# Autodesk Inventor assembly: full
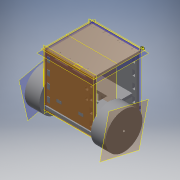
[picture p0: Inventor's stored thumbnail of the model, 180x180]
Saved by Autodesk Inventor 2018 (Build 220112000, 112)
## iProperties
Created: 2017-10-11
Part Number: full
Document SubType Name: Assembly
Designer: fabre
Author: fabre
## Documents named in this file (3)
- C:\Users\rfabre\Desktop\cubi\mechanics\full.iam
- C:\Users\rfabre\Desktop\cubi\mechanics\base.ipt
- C:\Users\rfabre\Desktop\cubi\mechanics\battery.ipt
## Components (2 placed, 2 different names)
1. base:1 — Mate:1, Mate:2, Mate:3
2. battery:1 — Mate:1, Mate:2, Mate:3
## Relationships (3: Mate 3)
- Mate:1: base:1 ↔ battery:1
- Mate:2: base:1 ↔ battery:1
- Mate:3: base:1 ↔ battery:1
